# Autodesk Inventor assembly: 2018 radiator analysis
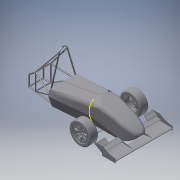
[picture p0: Inventor's stored thumbnail of the model, 180x180]
Saved by Autodesk Inventor 2018.2 (Build 222227000, 227)
## iProperties
Company: none
Created: 2018-02-25
Part Number: 2018 radiator analysis
Material: 一般
Description: CATIA V5 STEP Exchange
Document SubType Name: Assembly
Designer: ku_sk
Authority: none
Sending System: CATIA V5 STEP AP203
Preprocessor: CATIA Version 5 Release 17 (IN-10)
Title: Z:\各班フォルダ\2018\ボディ\カウル\AeroCAD2018\設計\2018 radiator analysis.stp
Author: none
## Documents named in this file (10)
- C:\Users\ku_sk\Documents\Inventor\AeroCAD2018\設計\Fr.wing\2018 radiator analysis.iam
- C:\Users\ku_sk\Documents\Inventor\AeroCAD2018\設計\Fr.wing\body\AssyTsutsui2018.iam
- C:\Users\ku_sk\Documents\Inventor\AeroCAD2018\設計\Fr.wing\body\SidePanel_Upper.ipt
- C:\Users\ku_sk\Documents\Inventor\AeroCAD2018\設計\Fr.wing\body\aaa.ipt
- C:\Users\ku_sk\Documents\Inventor\AeroCAD2018\設計\Fr.wing\Fr.wing.iam
- C:\Users\ku_sk\Documents\Inventor\AeroCAD2018\設計\Fr.wing\body\AssyTsutsui20181.iam
- C:\Users\ku_sk\Documents\Inventor\AeroCAD2018\設計\Fr.wing\body\SidePanel_Upper1.ipt
- C:\Users\ku_sk\Documents\Inventor\AeroCAD2018\設計\Fr.wing\body\aaa1.ipt
- C:\Users\ku_sk\Documents\Inventor\AeroCAD2018\設計\Fr.wing\Fr.wing2.iam
- C:\Users\ku_sk\Documents\Inventor\AeroCAD2018\設計\Fr.wing\frame2018.ipt
## Components (9 placed, 9 different names)
1. AssyTsutsui2018.1 [sub-assembly]
2. Part127.1
3. 2018Frontnose
4. Fr.wing:1 [sub-assembly] — メイト:1, メイト:2, メイト:3
5. AssyTsutsui20181:1 [sub-assembly]
6. SidePanel_Upper1:1
7. aaa1:1
8. Fr.wing2:1 [sub-assembly] — フラッシュ:1, メイト:2, メイト:3
9. frame2018:1 — フラッシュ:2, フラッシュ:3, フラッシュ:4
## Relationships (7: Flush 4, Mate 3)
- メイト:1 [Mate]: Fr.wing:1
- フラッシュ:1 [Flush]: Fr.wing2:1
- メイト:2 [Mate]: Fr.wing:1 ↔ Fr.wing2:1
- メイト:3 [Mate]: Fr.wing:1 ↔ Fr.wing2:1
- フラッシュ:2 [Flush]: frame2018:1
- フラッシュ:3 [Flush]: frame2018:1
- フラッシュ:4 [Flush]: frame2018:1
